# Autodesk Inventor assembly: HM-11
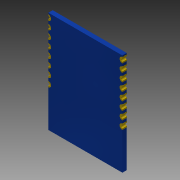
[picture p0: Inventor's stored thumbnail of the model, 180x180]
Saved by Autodesk Inventor 2013 (Build 170138000, 138)
## iProperties
Created: 2015-07-01
Part Number: HM-11
Document SubType Name: Assembly
Designer: terg
Author: terg
## Documents named in this file (5)
- C:\Users\terg\Projects\ModularElectronics\3D_models\Bluetooth_module\HM-11.iam
- C:\Users\terg\Projects\ModularElectronics\3D_models\Bluetooth_module\HM-11.ipt
- C:\Users\terg\Projects\ModularElectronics\3D_models\Components\0402_cap.ipt
- C:\Users\terg\Projects\ModularElectronics\3D_models\Components\0402_res.ipt
- C:\Users\terg\Projects\ModularElectronics\3D_models\Components\0603_cap.ipt
## Components (20 placed, 4 different names)
1. HM-11:1 — Zestawiający:1, Zestawiający:2, Zestawiający:3, Równoległy:1, Równoległy:2, Równoległy:3, Równoległy:4, Równoległy:5, Równoległy:6, Zestawiający:4, Zestawiający:5, Zestawiający:6, Zestawiający:7, Zestawiający:8, Zestawiający:9, Równoległy:7, Równoległy:8, Równoległy:9, Równoległy:10, Równoległy:11, Równoległy:12, Równoległy:16, Zestawiający:10, Zestawiający:11, Zestawiający:12, Zestawiający:13, Zestawiający:14, Zestawiający:15, Równoległy:17, Równoległy:18, Równoległy:24, Równoległy:25, Równoległy:26, Zestawiający:16, Zestawiający:17, Zestawiający:18, Zestawiający:19, Równoległy:27, Równoległy:28, Równoległy:29, Równoległy:30, Równoległy:33, Równoległy:34, Równoległy:35, Równoległy:36, Równoległy:38
2. 0402_cap:1 — Zestawiający:3, Równoległy:1, Równoległy:5
3. 0402_cap:2 — Zestawiający:2, Równoległy:3, Równoległy:6
4. 0402_cap:3 — Zestawiający:1, Równoległy:2, Równoległy:4
5. 0402_cap:4 — Zestawiający:4, Równoległy:7, Równoległy:38
6. 0402_cap:5 — Zestawiający:5, Równoległy:8, Równoległy:37
7. 0402_cap:6 — Zestawiający:6, Równoległy:9, Równoległy:15, Równoległy:16
8. 0402_cap:7 — Zestawiający:7, Równoległy:10, Równoległy:14, Równoległy:15
9. 0402_cap:8 — Zestawiający:8, Równoległy:11, Równoległy:13, Równoległy:14
10. 0402_cap:9 — Zestawiający:9, Równoległy:12, Równoległy:13
11. 0402_res:1 — Zestawiający:10, Równoległy:19, Równoległy:23
12. 0402_res:2 — Zestawiający:11, Równoległy:20, Równoległy:23, Równoległy:24, Równoległy:31
13. 0402_res:3 — Zestawiający:12, Równoległy:20, Równoległy:22, Równoległy:32, Równoległy:36
14. 0402_res:4 — Zestawiający:15, Równoległy:21, Równoległy:25
15. 0402_res:5 — Zestawiający:13, Równoległy:18, Równoległy:19, Równoległy:21, Równoległy:22
16. 0402_res:6 — Zestawiający:14, Równoległy:17, Równoległy:26
17. 0603_cap:1 — Zestawiający:16, Równoległy:33, Równoległy:34
18. 0402_res:7 — Zestawiający:17, Równoległy:27, Równoległy:28, Równoległy:37
19. 0402_res:8 — Zestawiający:18, Równoległy:29, Równoległy:31, Równoległy:35
20. 0402_cap:10 — Zestawiający:19, Równoległy:30, Równoległy:32
## Relationships (57: Flush 38, Mate 19)
- Zestawiający:1 [Mate]: HM-11:1 ↔ 0402_cap:3
- Zestawiający:2 [Mate]: HM-11:1 ↔ 0402_cap:2
- Zestawiający:3 [Mate]: HM-11:1 ↔ 0402_cap:1
- Równoległy:1 [Flush] (0.988 mm): HM-11:1 ↔ 0402_cap:1
- Równoległy:2 [Flush] (2.3 mm): HM-11:1 ↔ 0402_cap:3
- Równoległy:3 [Flush] (1.3 mm): HM-11:1 ↔ 0402_cap:2
- Równoległy:4 [Flush] (1.347 mm): HM-11:1 ↔ 0402_cap:3
- Równoległy:5 [Flush] (1.35 mm): HM-11:1 ↔ 0402_cap:1
- Równoległy:6 [Flush] (2 mm): HM-11:1 ↔ 0402_cap:2
- Zestawiający:4 [Mate]: HM-11:1 ↔ 0402_cap:4
- Zestawiający:5 [Mate]: HM-11:1 ↔ 0402_cap:5
- Zestawiający:6 [Mate]: HM-11:1 ↔ 0402_cap:6
- Zestawiający:7 [Mate]: HM-11:1 ↔ 0402_cap:7
- Zestawiający:8 [Mate]: HM-11:1 ↔ 0402_cap:8
- Zestawiający:9 [Mate]: HM-11:1 ↔ 0402_cap:9
- Równoległy:7 [Flush] (1.5 mm): HM-11:1 ↔ 0402_cap:4
- Równoległy:8 [Flush] (3 mm): HM-11:1 ↔ 0402_cap:5
- Równoległy:9 [Flush] (3.544 mm): HM-11:1 ↔ 0402_cap:6
- Równoległy:10 [Flush] (4.6 mm): HM-11:1 ↔ 0402_cap:7
- Równoległy:11 [Flush] (10.9 mm): HM-11:1 ↔ 0402_cap:8
- Równoległy:12 [Flush] (12 mm): HM-11:1 ↔ 0402_cap:9
- Równoległy:13 [Flush]: 0402_cap:8 ↔ 0402_cap:9
- Równoległy:14 [Flush]: 0402_cap:7 ↔ 0402_cap:8
- Równoległy:15 [Flush]: 0402_cap:6 ↔ 0402_cap:7
- Równoległy:16 [Flush] (9 mm): HM-11:1 ↔ 0402_cap:6
- Zestawiający:10 [Mate]: HM-11:1 ↔ 0402_res:1
- Zestawiający:11 [Mate]: HM-11:1 ↔ 0402_res:2
- Zestawiający:12 [Mate]: HM-11:1 ↔ 0402_res:3
- Zestawiający:13 [Mate]: HM-11:1 ↔ 0402_res:5
- Zestawiający:14 [Mate]: HM-11:1 ↔ 0402_res:6
- Zestawiający:15 [Mate]: HM-11:1 ↔ 0402_res:4
- Równoległy:17 [Flush] (3.439 mm): HM-11:1 ↔ 0402_res:6
- Równoległy:18 [Flush] (8.989 mm): HM-11:1 ↔ 0402_res:5
- Równoległy:19 [Flush] (0.024 mm): 0402_res:1 ↔ 0402_res:5
- Równoległy:20 [Flush] (0.017 mm): 0402_res:2 ↔ 0402_res:3
- Równoległy:21 [Flush] (-0.012 mm): 0402_res:4 ↔ 0402_res:5
- Równoległy:22 [Flush] (0.081 mm): 0402_res:3 ↔ 0402_res:5
- Równoległy:23 [Flush] (0.015 mm): 0402_res:1 ↔ 0402_res:2
- Równoległy:24 [Flush] (6.298 mm): HM-11:1 ↔ 0402_res:2
- Równoległy:25 [Flush] (3.195 mm): HM-11:1 ↔ 0402_res:4
- Równoległy:26 [Flush] (1.311 mm): HM-11:1 ↔ 0402_res:6
- Zestawiający:16 [Mate]: HM-11:1 ↔ 0603_cap:1
- Zestawiający:17 [Mate]: HM-11:1 ↔ 0402_res:7
- Zestawiający:18 [Mate]: HM-11:1 ↔ 0402_res:8
- Zestawiający:19 [Mate]: HM-11:1 ↔ 0402_cap:10
- Równoległy:27 [Flush] (1.5 mm): HM-11:1 ↔ 0402_res:7
- Równoległy:28 [Flush] (5.321 mm): HM-11:1 ↔ 0402_res:7
- Równoległy:29 [Flush] (6.69 mm): HM-11:1 ↔ 0402_res:8
- Równoległy:30 [Flush] (7.967 mm): HM-11:1 ↔ 0402_cap:10
- Równoległy:31 [Flush] (1.259 mm): 0402_res:2 ↔ 0402_res:8
- Równoległy:32 [Flush] (1.272 mm): 0402_res:3 ↔ 0402_cap:10
- Równoległy:33 [Flush] (2.812 mm): HM-11:1 ↔ 0603_cap:1
- Równoległy:34 [Flush] (2.575 mm): HM-11:1 ↔ 0603_cap:1
- Równoległy:35 [Flush] (11.425 mm): HM-11:1 ↔ 0402_res:8
- Równoległy:36 [Flush] (4.569 mm): HM-11:1 ↔ 0402_res:3
- Równoległy:37 [Flush] (0.017 mm): 0402_cap:5 ↔ 0402_res:7
- Równoległy:38 [Flush] (3.241 mm): HM-11:1 ↔ 0402_cap:4
